# Autodesk Inventor assembly: gateAssembly
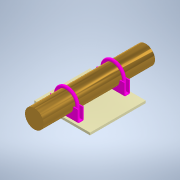
[picture p0: Inventor's stored thumbnail of the model, 180x180]
Saved by Autodesk Inventor 2020 (Build 240168000, 168)
## iProperties
Created: 2019-07-06
Part Number: gateAssembly
Document SubType Name: Assembly
Designer: steele
Author: steele
## Documents named in this file (4)
- C:\git\CAD-Development\robSteele\HouseProjects\automaticFrontGate\gateAssembly.iam
- C:\git\CAD-Development\robSteele\HouseProjects\automaticFrontGate\pipe.ipt
- C:\git\CAD-Development\robSteele\HouseProjects\automaticFrontGate\3042T870_CLAMPING U-BOLT.ipt
- C:\git\CAD-Development\robSteele\HouseProjects\automaticFrontGate\steelPlateForGate.ipt
## Components (4 placed, 3 different names)
1. pipe:1 — Mate:1, Flush:4, Mate:2, Mate:3, Mate:4, Mate:5, Mate:6, Flush:6
2. 3042T870_CLAMPING U-BOLT:1 — Flush:5, Mate:2, Mate:4
3. 3042T870_CLAMPING U-BOLT:2 — Flush:5, Mate:3, Mate:5, Mate:6
4. steelPlateForGate:1 — Mate:1, Flush:4, Flush:6
## Relationships (9: Mate 6, Flush 3)
- Mate:1 (-33.02 mm): pipe:1 ↔ steelPlateForGate:1
- Flush:4: pipe:1 ↔ steelPlateForGate:1
- Flush:5 (127 mm): 3042T870_CLAMPING U-BOLT:1 ↔ 3042T870_CLAMPING U-BOLT:2
- Mate:2: pipe:1 ↔ 3042T870_CLAMPING U-BOLT:1
- Mate:3: pipe:1 ↔ 3042T870_CLAMPING U-BOLT:2
- Mate:4: pipe:1 ↔ 3042T870_CLAMPING U-BOLT:1
- Mate:5: pipe:1 ↔ 3042T870_CLAMPING U-BOLT:2
- Mate:6 (88.9 mm): pipe:1 ↔ 3042T870_CLAMPING U-BOLT:2
- Flush:6 (-76.2 mm): pipe:1 ↔ steelPlateForGate:1
